# Autodesk Inventor assembly: frame
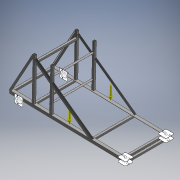
[picture p0: Inventor's stored thumbnail of the model, 180x180]
Saved by Autodesk Inventor 2018 (Build 220112000, 112)
## iProperties
Created: 2018-07-30
Part Number: frame
Document SubType Name: Assembly
Designer: Cole Tucker
Mass: 6614.31 g
Surface Area: 10202.1 cm^2
Volume: 2449.75 cm^3
Density: 2.7 g/cm^3
Author: Cole Tucker
## Documents named in this file (14)
- C:\Users\Cole Tucker\OneDrive\FRC-mxpProject\Cad\chassis\Inventor\frame.iam
- C:\Users\Cole Tucker\OneDrive\FRC-mxpProject\Cad\chassis\Inventor\22inSqTube.ipt
- C:\Users\Cole Tucker\OneDrive\FRC-mxpProject\Cad\chassis\Inventor\60in1.5Lch.ipt
- C:\Users\Cole Tucker\OneDrive\FRC-mxpProject\Cad\chassis\Inventor\bearingplaterear.ipt
- C:\Users\Cole Tucker\OneDrive\FRC-mxpProject\Cad\chassis\Inventor\24.8in1.0Lch.ipt
- C:\Users\Cole Tucker\OneDrive\FRC-mxpProject\Cad\chassis\Inventor\36in1.0Lch.ipt
- C:\Users\Cole Tucker\OneDrive\FRC-mxpProject\Cad\chassis\Inventor\22in1.0Lch.ipt
- C:\Users\Cole Tucker\OneDrive\FRC-mxpProject\Cad\chassis\Inventor\steeringPlate.ipt
- C:\Users\Cole Tucker\OneDrive\FRC-mxpProject\Cad\chassis\Inventor\frame\AIP\FEA\cl7sthen4.fins
- C:\Users\Cole Tucker\OneDrive\FRC-mxpProject\Cad\chassis\Inventor\frame\AIP\FEA\cl7sthen4.fsat
- C:\Users\Cole Tucker\OneDrive\FRC-mxpProject\Cad\chassis\Inventor\frame\AIP\FEA\cl7sthen4.ftes
- C:\Users\Cole Tucker\OneDrive\FRC-mxpProject\Cad\chassis\Inventor\frame\AIP\FEA\cl7sthen4.fwiz
- C:\Users\Cole Tucker\OneDrive\FRC-mxpProject\Cad\chassis\Inventor\frame\AIP\FEA\cl7stheow.fmsh
- C:\Users\Cole Tucker\OneDrive\FRC-mxpProject\Cad\chassis\Inventor\frame\AIP\FEA\cl7stheox.fres
## Components (24 placed, 7 different names)
1. 22inSqTube:1 — Flush:3, Mate:5, Mate:6, Mate:13, Mate:15, Mate:69, Mate:70
2. 22inSqTube:2 — Mate:1, Flush:1, Mate:2, Mate:3, Mate:4, Flush:2, Mate:14, Flush:15, Flush:16, Mate:63, Flush:17, Mate:65, Flush:18
3. 60in1.5Lch:1 — Mate:3, Mate:4, Flush:2, Flush:3, Mate:5, Mate:6, Mate:11, Mate:12, Mate:17, Flush:4, Mate:24, Mate:29, Mate:32, Mate:35, Mate:36, Mate:50, Mate:59, Flush:20, Flush:22, Mate:73, Mate:74
4. 60in1.5Lch:2 — Mate:1, Flush:1, Mate:2, Mate:7, Mate:8, Mate:9, Mate:10, Mate:16, Flush:5, Mate:25, Mate:28, Mate:30, Mate:34, Mate:37, Mate:49, Mate:60, Flush:19, Flush:21, Mate:71, Mate:72
5. 22inSqTube:3 — Mate:7, Mate:8, Mate:13, Flush:8, Flush:9
6. 22inSqTube:4 — Mate:9, Mate:11, Mate:15
7. 22inSqTube:5 — Mate:10, Mate:12, Mate:14
8. bearingplaterear:1 — Mate:16, Flush:5, Mate:70
9. bearingplaterear:2 — Mate:17, Flush:4, Mate:69
10. 22inSqTube:6 — Mate:25, Flush:9, Mate:31, Mate:39, Mate:41, Flush:10, Mate:43, Mate:53, Flush:21, Mate:67
11. 22inSqTube:7 — Mate:24, Flush:8, Mate:33, Mate:38, Mate:40, Mate:42, Mate:54, Mate:68, Flush:22
12. 24.8in1.0Lch:1 — Mate:28, Mate:30, Mate:31, Mate:67
13. 24.8in1.0Lch:2 — Mate:29, Mate:32, Mate:33, Mate:68
14. 36in1.0Lch:1 — Mate:34, Mate:37, Mate:39, Mate:41
15. 36in1.0Lch:2 — Mate:35, Mate:36, Mate:38, Mate:40
16. 22in1.0Lch:1 — Flush:10, Mate:42, Mate:43, Flush:13
17. 22inSqTube:8 — Mate:49, Mate:53, Mate:55, Mate:56, Mate:57, Mate:58, Flush:19
18. 22inSqTube:9 — Mate:50, Mate:54, Flush:20
19. 22in1.0Lch:3 — Flush:13, Mate:55, Mate:56, Flush:14
20. 22in1.0Lch:4 — Mate:57, Mate:58, Flush:14
21. steeringPlate:1 — Mate:59, Flush:16, Mate:73
22. steeringPlate:2 — Flush:15, Mate:60, Mate:71
23. steeringPlate:3 — Mate:65, Flush:18, Mate:74
24. steeringPlate:4 — Mate:63, Flush:17, Mate:72
## Relationships (73: Mate 55, Flush 18)
- Mate:1: 22inSqTube:2 ↔ 60in1.5Lch:2
- Flush:1: 22inSqTube:2 ↔ 60in1.5Lch:2
- Mate:2: 22inSqTube:2 ↔ 60in1.5Lch:2
- Mate:3: 22inSqTube:2 ↔ 60in1.5Lch:1
- Mate:4: 22inSqTube:2 ↔ 60in1.5Lch:1
- Flush:2: 22inSqTube:2 ↔ 60in1.5Lch:1
- Flush:3: 22inSqTube:1 ↔ 60in1.5Lch:1
- Mate:5: 22inSqTube:1 ↔ 60in1.5Lch:1
- Mate:6: 22inSqTube:1 ↔ 60in1.5Lch:1
- Mate:7: 60in1.5Lch:2 ↔ 22inSqTube:3
- Mate:8: 60in1.5Lch:2 ↔ 22inSqTube:3
- Mate:9: 60in1.5Lch:2 ↔ 22inSqTube:4
- Mate:10: 60in1.5Lch:2 ↔ 22inSqTube:5
- Mate:11: 60in1.5Lch:1 ↔ 22inSqTube:4
- Mate:12: 60in1.5Lch:1 ↔ 22inSqTube:5
- Mate:13 (254 mm): 22inSqTube:1 ↔ 22inSqTube:3
- Mate:14 (25.4 mm): 22inSqTube:2 ↔ 22inSqTube:5
- Mate:15 (1016 mm): 22inSqTube:1 ↔ 22inSqTube:4
- Mate:16: 60in1.5Lch:2 ↔ bearingplaterear:1
- Mate:17: 60in1.5Lch:1 ↔ bearingplaterear:2
- Flush:4: 60in1.5Lch:1 ↔ bearingplaterear:2
- Flush:5: 60in1.5Lch:2 ↔ bearingplaterear:1
- Mate:24: 60in1.5Lch:1 ↔ 22inSqTube:7
- Mate:25: 60in1.5Lch:2 ↔ 22inSqTube:6
- Flush:8 (12.7 mm): 22inSqTube:3 ↔ 22inSqTube:7
- Flush:9 (12.7 mm): 22inSqTube:3 ↔ 22inSqTube:6
- Mate:28: 60in1.5Lch:2 ↔ 24.8in1.0Lch:1
- Mate:29: 60in1.5Lch:1 ↔ 24.8in1.0Lch:2
- Mate:30: 60in1.5Lch:2 ↔ 24.8in1.0Lch:1
- Mate:31: 22inSqTube:6 ↔ 24.8in1.0Lch:1
- Mate:32: 60in1.5Lch:1 ↔ 24.8in1.0Lch:2
- Mate:33: 22inSqTube:7 ↔ 24.8in1.0Lch:2
- Mate:34: 60in1.5Lch:2 ↔ 36in1.0Lch:1
- Mate:35: 60in1.5Lch:1 ↔ 36in1.0Lch:2
- Mate:36: 60in1.5Lch:1 ↔ 36in1.0Lch:2
- Mate:37: 60in1.5Lch:2 ↔ 36in1.0Lch:1
- Mate:38: 22inSqTube:7 ↔ 36in1.0Lch:2
- Mate:39: 22inSqTube:6 ↔ 36in1.0Lch:1
- Mate:40 (38.1 mm): 22inSqTube:7 ↔ 36in1.0Lch:2
- Mate:41 (38.1 mm): 22inSqTube:6 ↔ 36in1.0Lch:1
- Flush:10 (76.2 mm): 22inSqTube:6 ↔ 22in1.0Lch:1
- Mate:42: 22inSqTube:7 ↔ 22in1.0Lch:1
- Mate:43: 22inSqTube:6 ↔ 22in1.0Lch:1
- Mate:49: 60in1.5Lch:2 ↔ 22inSqTube:8
- Mate:50: 60in1.5Lch:1 ↔ 22inSqTube:9
- Mate:53 (203.2 mm): 22inSqTube:6 ↔ 22inSqTube:8
- Mate:54 (203.2 mm): 22inSqTube:7 ↔ 22inSqTube:9
- Flush:13 (50.8 mm): 22in1.0Lch:1 ↔ 22in1.0Lch:3
- Mate:55: 22inSqTube:8 ↔ 22in1.0Lch:3
- Mate:56: 22inSqTube:8 ↔ 22in1.0Lch:3
- Mate:57: 22inSqTube:8 ↔ 22in1.0Lch:4
- Mate:58: 22inSqTube:8 ↔ 22in1.0Lch:4
- Flush:14 (304.8 mm): 22in1.0Lch:3 ↔ 22in1.0Lch:4
- Mate:59: 60in1.5Lch:1 ↔ steeringPlate:1
- Flush:15: 22inSqTube:2 ↔ steeringPlate:2
- Flush:16: 22inSqTube:2 ↔ steeringPlate:1
- Mate:60: 60in1.5Lch:2 ↔ steeringPlate:2
- Mate:63: 22inSqTube:2 ↔ steeringPlate:4
- Flush:17: 22inSqTube:2 ↔ steeringPlate:4
- Mate:65: 22inSqTube:2 ↔ steeringPlate:3
- Flush:18: 22inSqTube:2 ↔ steeringPlate:3
- Flush:19: 60in1.5Lch:2 ↔ 22inSqTube:8
- Flush:20: 60in1.5Lch:1 ↔ 22inSqTube:9
- Flush:21: 60in1.5Lch:2 ↔ 22inSqTube:6
- Mate:67: 22inSqTube:6 ↔ 24.8in1.0Lch:1
- Mate:68: 22inSqTube:7 ↔ 24.8in1.0Lch:2
- Mate:69 (-127 mm): 22inSqTube:1 ↔ bearingplaterear:2
- Mate:70 (-127 mm): 22inSqTube:1 ↔ bearingplaterear:1
- Flush:22: 60in1.5Lch:1 ↔ 22inSqTube:7
- Mate:71 (19.05 mm): 60in1.5Lch:2 ↔ steeringPlate:2
- Mate:72 (19.05 mm): 60in1.5Lch:2 ↔ steeringPlate:4
- Mate:73 (19.05 mm): 60in1.5Lch:1 ↔ steeringPlate:1
- Mate:74 (19.05 mm): 60in1.5Lch:1 ↔ steeringPlate:3
## Named parameters: sa_0 = -0, sa_1 = -133447, sa_2 = -2.22411e-11
note: some values were not read from the file. Shown as the stored number, unit unknown: "sa_0", "sa_1", "sa_2".
